# Autodesk Inventor assembly: !back_clamp
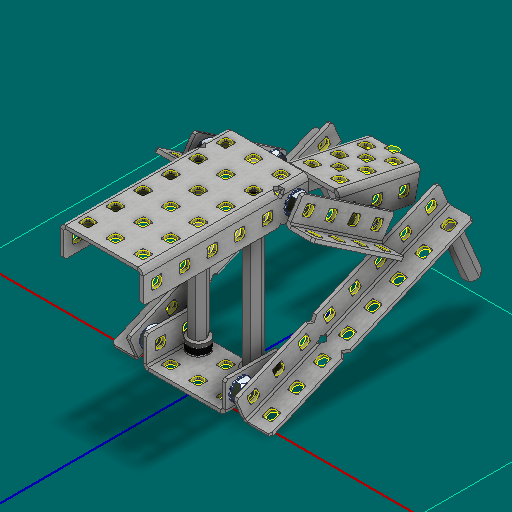
[picture p0: Inventor's stored thumbnail of the model, 512x512]
Saved by Autodesk Inventor 2025 (Build 290162000, 162)
## iProperties
Created: 2024-10-05
Part Number: !back_clamp
Document SubType Name: Assembly
Designer: averey
Author: averey
## Documents named in this file (18)
- C:\Users\avere\vex_robotics_high_stakes\hardware\cad\bots\high_stakes_v2\back_clamp\!back_clamp.iam
- C:\Users\avere\vex_robotics_high_stakes\hardware\cad\robpros_cad_lib\Structure\C Channel\Aluminum 1x3x1\Alu C 1x3x1x6.ipt
- C:\Users\avere\vex_robotics_high_stakes\hardware\cad\robpros_cad_lib\Structure\C Channel\Aluminum 1x3x1\Alu C 1x3x1x2.ipt
- C:\Users\avere\vex_robotics_high_stakes\hardware\cad\robpros_cad_lib\Structure\Standoff\Standoff 2.50.ipt
- C:\Users\avere\vex_robotics_high_stakes\hardware\cad\robpros_cad_lib\Structure\Standoff.ipt
- C:\Users\avere\vex_robotics_high_stakes\hardware\cad\robpros_cad_lib\Motion\Spacers\Spacer Nylon .375 OD\NSpacer .375 OD x .125.ipt
- C:\Users\avere\vex_robotics_high_stakes\hardware\cad\robpros_cad_lib\Motion\Spacers\Spacer Nylon .375 OD.ipt
- C:\Users\avere\vex_robotics_high_stakes\hardware\cad\robpros_cad_lib\Motion\Spacers\Washer Steel\SWasher .375 OD x .031250.ipt
- C:\Users\avere\vex_robotics_high_stakes\hardware\cad\robpros_cad_lib\Motion\Spacers\Washer Steel.ipt
- C:\Users\avere\vex_robotics_high_stakes\hardware\cad\robpros_cad_lib\Motion\Spacers\Washer Steel\SWasher .375 OD x .062500.ipt
- C:\Users\avere\vex_robotics_high_stakes\hardware\cad\robpros_cad_lib\Motion\Spacers\Washer Steel\SWasher .375 OD x .015625.ipt
- C:\Users\avere\vex_robotics_high_stakes\hardware\cad\robpros_cad_lib\Structure\Hardware\Nut Keps.ipt
- C:\Users\avere\vex_robotics_high_stakes\hardware\cad\robpros_cad_lib\Structure\Angle\Aluminum 1x1\Alu Angle 1x1x5.ipt
- C:\Users\avere\vex_robotics_high_stakes\hardware\cad\robpros_cad_lib\Structure\C Channel\Aluminum 1x2x1\Alu C 1x2x1x4.ipt
- C:\Users\avere\vex_robotics_high_stakes\hardware\cad\robpros_cad_lib\Structure\Angle\Aluminum 1x1\Alu Angle 1x1x8.ipt
- C:\Users\avere\vex_robotics_high_stakes\hardware\cad\robpros_cad_lib\Structure\Angle\Aluminum 1x1\Alu Angle 1x1x4.ipt
- C:\Users\avere\vex_robotics_high_stakes\hardware\cad\robpros_cad_lib\Structure\Standoff\Standoff 1.00.ipt
- C:\Users\avere\vex_robotics_high_stakes\hardware\cad\robpros_cad_lib\Structure\C Channel\Aluminum 1x2x1\Alu C 1x2x1x3.ipt
## Components (33 placed, 14 different names)
1. Alu C 1x3x1x6:1 — Insert:23, Insert:24
2. Alu C 1x3x1x2:1 — Mate:2, Insert:30, Insert:38
3. NSpacer .375 OD x .125:1
4. NSpacer .375 OD x .125:2
5. SWasher .375 OD x .031250:1
6. SWasher .375 OD x .062500:2
7. SWasher .375 OD x .062500:3 — Insert:35
8. SWasher .375 OD x .015625:4
9. SWasher .375 OD x .062500:7
10. NSpacer .375 OD x .125:5
11. NSpacer .375 OD x .125:6
12. SWasher .375 OD x .031250:9
13. SWasher .375 OD x .062500:10 — Insert:34
14. SWasher .375 OD x .062500:11
15. SWasher .375 OD x .015625:12
16. Nut Keps:1 — Insert:24, Insert:26
17. Nut Keps:2 — Insert:23, Insert:25
18. Alu Angle 1x1x5:1 — Insert:26, Mate:3, Insert:33, Insert:37, Mate:6
19. Alu Angle 1x1x5:2 — Insert:25, Mate:3, Insert:32, Insert:36
20. Alu C 1x2x1x4:1 — Mate:4, Mate:8, Insert:39, Insert:42, Mate:10
21. Nut Keps:3 — Insert:32, Mate:5, Insert:39
22. Nut Keps:5 — Insert:33
23. Alu Angle 1x1x8:2 — Insert:31, Mate:4, Insert:41
24. Nut Keps:6 — Insert:30, Insert:31
25. Standoff 2.50:1 — Insert:35
26. Standoff 2.50:2 — Insert:34
27. Alu Angle 1x1x4:1 — Insert:36, Mate:5, Flush:1, Mate:9
28. Alu Angle 1x1x4:2 — Insert:37, Mate:6
29. Alu Angle 1x1x8:3 — Mate:7, Flush:1, Mate:8, Insert:40, Mate:9
30. Nut Keps:7 — Insert:38, Mate:7
31. Standoff 1.00:3 — Insert:40
32. Standoff 1.00:4 — Insert:41
33. Alu C 1x2x1x3:1 — Insert:42, Mate:10
## Relationships (39: Insert 28, Mate 10, Flush 1)
- [Insert]: NSpacer .375 OD x .125:1 ↔ SWasher .375 OD x .062500:2
- [Insert]: NSpacer .375 OD x .125:2 ↔ SWasher .375 OD x .062500:3
- [Insert]: NSpacer .375 OD x .125:1 ↔ SWasher .375 OD x .015625:4
- [Insert]: NSpacer .375 OD x .125:2 ↔ SWasher .375 OD x .031250:1
- [Insert]: Alu C 1x3x1x2:1 ↔ SWasher .375 OD x .031250:1
- [Insert]: NSpacer .375 OD x .125:5 ↔ SWasher .375 OD x .062500:10
- [Insert]: NSpacer .375 OD x .125:6 ↔ SWasher .375 OD x .062500:11
- [Insert]: NSpacer .375 OD x .125:5 ↔ SWasher .375 OD x .015625:12
- [Insert]: NSpacer .375 OD x .125:6 ↔ SWasher .375 OD x .031250:9
- [Insert]: Alu C 1x3x1x2:1 ↔ SWasher .375 OD x .015625:12
- [Insert] (74.1934 mm): Alu C 1x3x1x6:1 ↔ Alu C 1x3x1x2:1
- [Mate]: Alu C 1x3x1x6:1 ↔ Alu C 1x3x1x2:1
- Mate:2: Alu C 1x3x1x2:1
- Insert:23: Alu C 1x3x1x6:1 ↔ Nut Keps:2
- Insert:24: Alu C 1x3x1x6:1 ↔ Nut Keps:1
- Insert:25 (1.016 mm): Nut Keps:2 ↔ Alu Angle 1x1x5:2
- Insert:26 (1.016 mm): Nut Keps:1 ↔ Alu Angle 1x1x5:1
- Mate:3: Alu Angle 1x1x5:1 ↔ Alu Angle 1x1x5:2
- Insert:30: Alu C 1x3x1x2:1 ↔ Nut Keps:6
- Insert:31 (1.016 mm): Alu Angle 1x1x8:2 ↔ Nut Keps:6
- Mate:4: Alu C 1x2x1x4:1 ↔ Alu Angle 1x1x8:2
- Insert:32: Alu Angle 1x1x5:2 ↔ Nut Keps:3
- Insert:33: Alu Angle 1x1x5:1 ↔ Nut Keps:5
- Insert:34: SWasher .375 OD x .062500:10 ↔ Standoff 2.50:2
- Insert:35: SWasher .375 OD x .062500:3 ↔ Standoff 2.50:1
- Insert:36: Alu Angle 1x1x5:2 ↔ Alu Angle 1x1x4:1
- Mate:5: Nut Keps:3 ↔ Alu Angle 1x1x4:1
- Insert:37: Alu Angle 1x1x5:1 ↔ Alu Angle 1x1x4:2
- Mate:6: Alu Angle 1x1x5:1 ↔ Alu Angle 1x1x4:2
- Insert:38: Alu C 1x3x1x2:1 ↔ Nut Keps:7
- Mate:7: Alu Angle 1x1x8:3 ↔ Nut Keps:7
- Flush:1: Alu Angle 1x1x4:1 ↔ Alu Angle 1x1x8:3
- Mate:8: Alu C 1x2x1x4:1 ↔ Alu Angle 1x1x8:3
- Insert:39 (7.366 mm): Alu C 1x2x1x4:1 ↔ Nut Keps:3
- Insert:40: Alu Angle 1x1x8:3 ↔ Standoff 1.00:3
- Insert:41: Alu Angle 1x1x8:2 ↔ Standoff 1.00:4
- Mate:9: Alu Angle 1x1x4:1 ↔ Alu Angle 1x1x8:3
- Insert:42: Alu C 1x2x1x4:1 ↔ Alu C 1x2x1x3:1
- Mate:10: Alu C 1x2x1x4:1 ↔ Alu C 1x2x1x3:1
## Named parameters: d20_d7 = 0 mm, d22_d9 = 0 mm, d24_d11 = 0 mm, d25_d12 = 0 mm
